# Autodesk Inventor assembly: tube
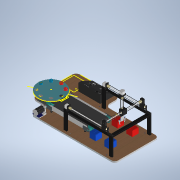
[picture p0: Inventor's stored thumbnail of the model, 180x180]
Saved by Autodesk Inventor 2021 (Build 250183000, 183)
## iProperties
Created: 2025-10-28
Part Number: tube
Document SubType Name: Assembly
Designer: MichaelHanyShawkyHab
Author: MichaelHanyShawkyHab
## Documents named in this file (14)
- C:\Users\MichaelHanyShawkyHab\Downloads\tube\tube.iam
- C:\Users\MichaelHanyShawkyHab\Downloads\tube\FEEDER_1.ipt
- C:\Users\MichaelHanyShawkyHab\Downloads\tube\Z_AXIS.ipt
- C:\Users\MichaelHanyShawkyHab\Downloads\tube\Y_AXIS.ipt
- C:\Users\MichaelHanyShawkyHab\Downloads\tube\X_AXIS.ipt
- C:\Users\MichaelHanyShawkyHab\Downloads\tube\base_1.ipt
- C:\Users\MichaelHanyShawkyHab\Downloads\tube\Gear.ipt
- C:\Users\MichaelHanyShawkyHab\Downloads\tube\Holder.ipt
- C:\Users\MichaelHanyShawkyHab\Downloads\tube\Stand.ipt
- C:\Users\MichaelHanyShawkyHab\Downloads\tube\Gear_MIR.ipt
- C:\Users\MichaelHanyShawkyHab\Downloads\tube\Holder_MIR.ipt
- C:\Users\MichaelHanyShawkyHab\Downloads\tube\Stand_MIR.ipt
- C:\Users\MichaelHanyShawkyHab\Downloads\tube\LID_Product_1.ipt
- C:\Users\MichaelHanyShawkyHab\Downloads\tube\base_product_1.ipt
## Components (15 placed, 13 different names)
1. FEEDER_1:1 — Rotational:1
2. Z_AXIS:1 — Mate:5, Mate:6, Rotational:4, Rotational:5, Rotational:8, Rotational:9
3. Y_AXIS:1 — Mate:3, Mate:4, Mate:5, Mate:6
4. X_AXIS:1 — Mate:1, Mate:2, Mate:3, Mate:4
5. base_1:1 — Mate:1, Mate:2, Rotational:1
6. Gear:1 — Rotational:3, Rotational:4
7. Holder:1 — Rotational:2, Rotational:3
8. Stand:1 — Rotational:2, Rotational:5
9. Gear_MIR:1 — Rotational:6, Rotational:8
10. Holder_MIR:1 — Rotational:6, Rotational:7
11. Stand_MIR:1 — Rotational:7, Rotational:9
12. LID_Product_1:1
13. base_product_1:1
14. LID_Product_1:2
15. base_product_1:2
## Relationships (15: RevoluteJoint 9, Mate 6)
- Mate:1: X_AXIS:1 ↔ base_1:1
- Mate:2: X_AXIS:1 ↔ base_1:1
- Mate:3: Y_AXIS:1 ↔ X_AXIS:1
- Mate:4: Y_AXIS:1 ↔ X_AXIS:1
- Mate:5: Z_AXIS:1 ↔ Y_AXIS:1
- Mate:6: Z_AXIS:1 ↔ Y_AXIS:1
- Rotational:1 [RevoluteJoint] (-10 mm): FEEDER_1:1 ↔ base_1:1
- Rotational:2 [RevoluteJoint]: Holder:1 ↔ Stand:1
- Rotational:3 [RevoluteJoint]: Gear:1 ↔ Holder:1
- Rotational:4 [RevoluteJoint]: Z_AXIS:1 ↔ Gear:1
- Rotational:5 [RevoluteJoint]: Z_AXIS:1 ↔ Stand:1
- Rotational:6 [RevoluteJoint]: Gear_MIR:1 ↔ Holder_MIR:1
- Rotational:7 [RevoluteJoint]: Holder_MIR:1 ↔ Stand_MIR:1
- Rotational:8 [RevoluteJoint]: Z_AXIS:1 ↔ Gear_MIR:1
- Rotational:9 [RevoluteJoint]: Z_AXIS:1 ↔ Stand_MIR:1
